# Autodesk Inventor assembly: Конвейр сборка
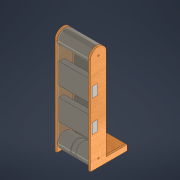
[picture p0: Inventor's stored thumbnail of the model, 180x180]
Saved by Autodesk Inventor 2022 (Build 260153000, 153)
## iProperties
Created: 2023-02-18
Part Number: Конвейр сборка
Document SubType Name: Assembly
Designer: Глеб
Author: Глеб
## Documents named in this file (7)
- C:\Users\Глеб\Documents\Inventor\Файлы Inventor\Конвейр сборка.iam
- C:\Users\Глеб\Documents\Inventor\Файлы Inventor\Стенка конвейера.ipt
- C:\Users\Глеб\Documents\Inventor\Файлы Inventor\Подставка для двигателя и драйвера.ipt
- C:\Users\Глеб\Documents\Inventor\Файлы Inventor\Вал конвейера.ipt
- C:\Users\Глеб\Documents\Inventor\Файлы Inventor\Вал конвейера 2.ipt
- C:\Users\Глеб\Documents\Inventor\Файлы Inventor\Стенкка для ковнейера.ipt
- C:\Users\Глеб\Documents\Inventor\Файлы Inventor\Лента конвейера.ipt
## Components (8 placed, 6 different names)
1. Стенка конвейера:1 — Совмещение:7, Совмещение:8, Совмещение:9, Совмещение:10, Заподлицо:2, Совмещение:16, Совмещение:17, Совмещение:22
2. Стенка конвейера:2 — Заподлицо:1, Совмещение:11, Совмещение:12, Совмещение:13, Совмещение:14, Совмещение:15, Совмещение:18, Совмещение:19, Совмещение:20, Заподлицо:3, Совмещение:21
3. Вал конвейера:1 — Совмещение:7, Совмещение:8
4. Вал конвейера 2:1 — Совмещение:9, Совмещение:10
5. Подставка для двигателя и драйвера:1 — Заподлицо:1, Совмещение:11, Совмещение:12
6. Подставка для двигателя и драйвера:2 — Совмещение:13, Совмещение:14, Совмещение:15, Заподлицо:2, Совмещение:16, Совмещение:17
7. Стенкка для ковнейера:1 — Совмещение:18, Совмещение:19, Совмещение:20
8. Лента конвейера:1 — Заподлицо:3, Совмещение:21, Совмещение:22
## Relationships (19: Mate 16, Flush 3)
- Совмещение:7 [Mate]: Стенка конвейера:1 ↔ Вал конвейера:1
- Совмещение:8 [Mate]: Стенка конвейера:1 ↔ Вал конвейера:1
- Совмещение:9 [Mate]: Стенка конвейера:1 ↔ Вал конвейера 2:1
- Совмещение:10 [Mate]: Стенка конвейера:1 ↔ Вал конвейера 2:1
- Заподлицо:1 [Flush]: Стенка конвейера:2 ↔ Подставка для двигателя и драйвера:1
- Совмещение:11 [Mate]: Стенка конвейера:2 ↔ Подставка для двигателя и драйвера:1
- Совмещение:12 [Mate]: Стенка конвейера:2 ↔ Подставка для двигателя и драйвера:1
- Совмещение:13 [Mate]: Стенка конвейера:2 ↔ Подставка для двигателя и драйвера:2
- Совмещение:14 [Mate]: Стенка конвейера:2 ↔ Подставка для двигателя и драйвера:2
- Совмещение:15 [Mate]: Стенка конвейера:2 ↔ Подставка для двигателя и драйвера:2
- Заподлицо:2 [Flush]: Стенка конвейера:1 ↔ Подставка для двигателя и драйвера:2
- Совмещение:16 [Mate]: Стенка конвейера:1 ↔ Подставка для двигателя и драйвера:2
- Совмещение:17 [Mate]: Стенка конвейера:1 ↔ Подставка для двигателя и драйвера:2
- Совмещение:18 [Mate]: Стенка конвейера:2 ↔ Стенкка для ковнейера:1
- Совмещение:19 [Mate]: Стенка конвейера:2 ↔ Стенкка для ковнейера:1
- Совмещение:20 [Mate]: Стенка конвейера:2 ↔ Стенкка для ковнейера:1
- Заподлицо:3 [Flush]: Стенка конвейера:2 ↔ Лента конвейера:1
- Совмещение:21 [Mate]: Стенка конвейера:2 ↔ Лента конвейера:1
- Совмещение:22 [Mate]: Стенка конвейера:1 ↔ Лента конвейера:1
